# Autodesk Inventor assembly: BD Gearbox and Bracket Assy 4
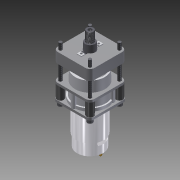
[picture p0: Inventor's stored thumbnail of the model, 180x180]
Saved by Autodesk Inventor 2012 (Build 160160000, 160)
## iProperties
Created: 2012-07-05
Part Number: BD Gearbox and Bracket Assy 4
Document SubType Name: Assembly
Designer: Bruce
Author: Bruce
## Documents named in this file (8)
- C:\Users\Bryce\Dropbox\Inventor Design Project Files\Independent Swerves\Imported Components\BD Gearbox and Bracket Assy 4.iam
- C:\Users\Bryce\Dropbox\Inventor Design Project Files\Independent Swerves\Imported Components\BD Drill motor assembly.iam
- C:\Users\Bryce\Dropbox\Inventor Design Project Files\Independent Swerves\Imported Components\BD gearbox mount block motor ring.ipt
- C:\Users\Bryce\Dropbox\Inventor Design Project Files\Independent Swerves\Imported Components\BD gearbox mount center ring.ipt
- C:\Users\Bryce\Dropbox\Inventor Design Project Files\Independent Swerves\Imported Components\Spacers BD gearbox back to ctr.ipt
- C:\Users\Bryce\Dropbox\Inventor Design Project Files\Independent Swerves\Imported Components\Bolt 8-32 gearbox mount TL.ipt
- C:\Users\Bryce\Dropbox\Inventor Design Project Files\Independent Swerves\Imported Components\Spring BD drill motor.ipt
- C:\Users\Bryce\Dropbox\Inventor Design Project Files\Independent Swerves\Imported Components\BD gearbox mount block 2.ipt
## Components (13 placed, 7 different names)
1. BD gearbox mount block motor ring:1 — Mate:5, Mate:7, Mate:8, Insert:1, Insert:2, Insert:3, Mate:12, Mate:15, Mate:17, Mate:19, Mate:22, Mate:23
2. BD Drill motor assembly:1 [sub-assembly] — Mate:5, Mate:22, Mate:23, Mate:27, Mate:28
3. Bolt 8-32 gearbox mount TL:1 — Mate:7, Mate:8, Mate:9, Mate:14, Mate:29
4. Bolt 8-32 gearbox mount TL:2 — Insert:3, Mate:11
5. Bolt 8-32 gearbox mount TL:3 — Insert:2, Mate:16, Mate:30
6. Bolt 8-32 gearbox mount TL:4 — Insert:1, Mate:10, Mate:18
7. BD gearbox mount center ring:1 — Mate:9, Mate:10, Mate:13
8. Spacers BD gearbox back to ctr:1 — Mate:11, Mate:12, Mate:13
9. Spacers BD gearbox back to ctr:2 — Mate:14, Mate:15
10. Spacers BD gearbox back to ctr:3 — Mate:16, Mate:17
11. Spacers BD gearbox back to ctr:4 — Mate:18, Mate:19
12. BD gearbox mount block 2:1 — Mate:28, Mate:29, Mate:30
13. Spring BD drill motor:1 — Mate:27
## Relationships (23: Mate 20, Insert 3)
- Mate:5: BD gearbox mount block motor ring:1 ↔ BD Drill motor assembly:1
- Mate:7: BD gearbox mount block motor ring:1 ↔ Bolt 8-32 gearbox mount TL:1
- Mate:8: BD gearbox mount block motor ring:1 ↔ Bolt 8-32 gearbox mount TL:1
- Insert:1: BD gearbox mount block motor ring:1 ↔ Bolt 8-32 gearbox mount TL:4
- Insert:2: BD gearbox mount block motor ring:1 ↔ Bolt 8-32 gearbox mount TL:3
- Insert:3: BD gearbox mount block motor ring:1 ↔ Bolt 8-32 gearbox mount TL:2
- Mate:9: Bolt 8-32 gearbox mount TL:1 ↔ BD gearbox mount center ring:1
- Mate:10: Bolt 8-32 gearbox mount TL:4 ↔ BD gearbox mount center ring:1
- Mate:11: Bolt 8-32 gearbox mount TL:2 ↔ Spacers BD gearbox back to ctr:1
- Mate:12: BD gearbox mount block motor ring:1 ↔ Spacers BD gearbox back to ctr:1
- Mate:13: BD gearbox mount center ring:1 ↔ Spacers BD gearbox back to ctr:1
- Mate:14: Bolt 8-32 gearbox mount TL:1 ↔ Spacers BD gearbox back to ctr:2
- Mate:15: BD gearbox mount block motor ring:1 ↔ Spacers BD gearbox back to ctr:2
- Mate:16: Bolt 8-32 gearbox mount TL:3 ↔ Spacers BD gearbox back to ctr:3
- Mate:17: BD gearbox mount block motor ring:1 ↔ Spacers BD gearbox back to ctr:3
- Mate:18: Bolt 8-32 gearbox mount TL:4 ↔ Spacers BD gearbox back to ctr:4
- Mate:19: BD gearbox mount block motor ring:1 ↔ Spacers BD gearbox back to ctr:4
- Mate:22: BD gearbox mount block motor ring:1 ↔ BD Drill motor assembly:1
- Mate:23: BD gearbox mount block motor ring:1 ↔ BD Drill motor assembly:1
- Mate:27: BD Drill motor assembly:1 ↔ Spring BD drill motor:1
- Mate:28: BD Drill motor assembly:1 ↔ BD gearbox mount block 2:1
- Mate:29: Bolt 8-32 gearbox mount TL:1 ↔ BD gearbox mount block 2:1
- Mate:30: Bolt 8-32 gearbox mount TL:3 ↔ BD gearbox mount block 2:1
